# Autodesk Inventor assembly: Pogo_Set1
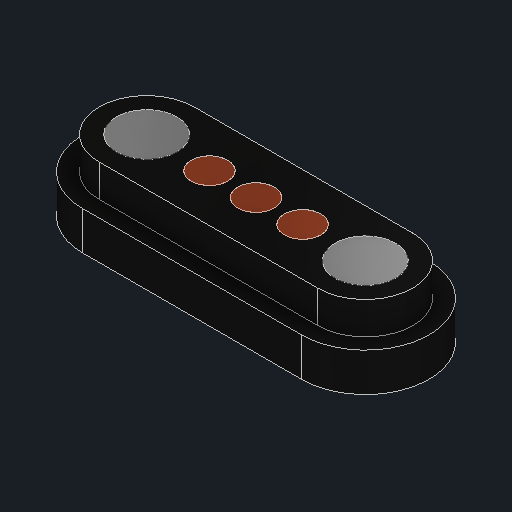
[picture p0: Inventor's stored thumbnail of the model, 512x512]
Saved by Autodesk Inventor 2026 (Build 300175000, 175)
## iProperties
Created: 2025-04-17
Part Number: Pogo_Set1
Document SubType Name: Assembly
Designer: ct_vi
Author: ct_vi
## Documents named in this file (4)
- C:\Users\ct_vi\Documents\Capstone_Research_3D_Files\Pogo_Set1.iam
- C:\Users\ct_vi\Documents\Capstone_Research_3D_Files\Pogo_Pin1.ipt
- C:\Users\ct_vi\Documents\Capstone_Research_3D_Files\Pogo1.ipt
- C:\Users\ct_vi\Documents\Capstone_Research_3D_Files\Pogo_Magnet1.ipt
## Components (4 placed, 3 different names)
1. Pogo_Pin1:1 — Mate:1, Mate:2
2. Pogo1:1 — Mate:1, Mate:2, Flush:1, Mate:3, Mate:4, Mate:5
3. Pogo_Magnet1:1 — Flush:1, Mate:5
4. Pogo_Magnet1:2 — Mate:3, Mate:4
## Relationships (6: Mate 5, Flush 1)
- Mate:1: Pogo_Pin1:1 ↔ Pogo1:1
- Mate:2: Pogo_Pin1:1 ↔ Pogo1:1
- Flush:1: Pogo1:1 ↔ Pogo_Magnet1:1
- Mate:3: Pogo1:1 ↔ Pogo_Magnet1:2
- Mate:4: Pogo1:1 ↔ Pogo_Magnet1:2
- Mate:5: Pogo1:1 ↔ Pogo_Magnet1:1
